# Autodesk Inventor assembly: auto
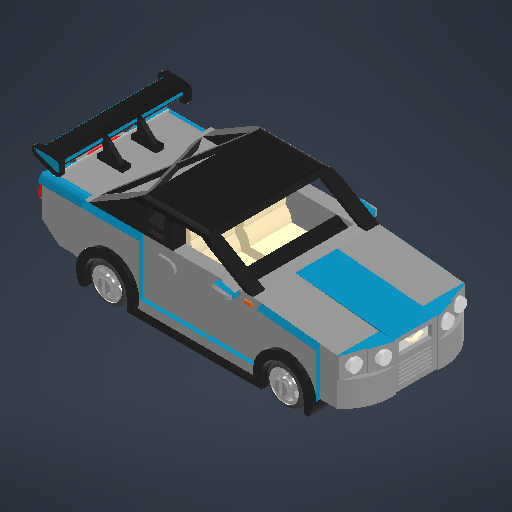
[picture p0: Inventor's stored thumbnail of the model, 512x512]
Saved by Autodesk Inventor 2026.2 (Build 302298000, 298)
## iProperties
Created: 2026-08-18
Part Number: auto
Document SubType Name: Assembly
Designer: wojsl
Author: wojsl
## Documents named in this file (6)
- C:\Users\wojsl\OneDrive\Pulpit\cad\samochód\auto.iam
- C:\Users\wojsl\OneDrive\Pulpit\cad\samochód\main.ipt
- C:\Users\wojsl\OneDrive\Pulpit\cad\samochód\main2.ipt
- C:\Users\wojsl\OneDrive\Pulpit\cad\samochód\dach.ipt
- C:\Users\wojsl\OneDrive\Pulpit\cad\samochód\opona.ipt
- C:\Users\wojsl\OneDrive\Pulpit\cad\samochód\fotel.ipt
## Components (9 placed, 5 different names)
1. main:1 — Wstawiające:1, Wstawiające:2, Wstawiające:3, Wstawiające:4, Wstawiające:5, Wstawiające:6, Wstawiające:7, Wstawiające:8, Wstawiające:9, Wstawiające:10, Wstawiające:11, Wstawiające:12
2. main2:1 — Wstawiające:1, Wstawiające:2
3. dach:1 — Wstawiające:3, Wstawiające:4
4. opona:1 — Wstawiające:7
5. opona:2 — Wstawiające:8
6. opona:3 — Wstawiające:6
7. opona:4 — Wstawiające:5
8. fotel:1 — Wstawiające:9, Wstawiające:10
9. fotel:2 — Wstawiające:11, Wstawiające:12
## Relationships (12: Insert 12)
- Wstawiające:1 [Insert]: main:1 ↔ main2:1
- Wstawiające:2 [Insert]: main:1 ↔ main2:1
- Wstawiające:3 [Insert]: main:1 ↔ dach:1
- Wstawiające:4 [Insert]: main:1 ↔ dach:1
- Wstawiające:5 [Insert]: main:1 ↔ opona:4
- Wstawiające:6 [Insert]: main:1 ↔ opona:3
- Wstawiające:7 [Insert]: main:1 ↔ opona:1
- Wstawiające:8 [Insert]: main:1 ↔ opona:2
- Wstawiające:9 [Insert]: main:1 ↔ fotel:1
- Wstawiające:10 [Insert]: main:1 ↔ fotel:1
- Wstawiające:11 [Insert]: main:1 ↔ fotel:2
- Wstawiające:12 [Insert]: main:1 ↔ fotel:2
